# Autodesk Inventor assembly: Złożenie
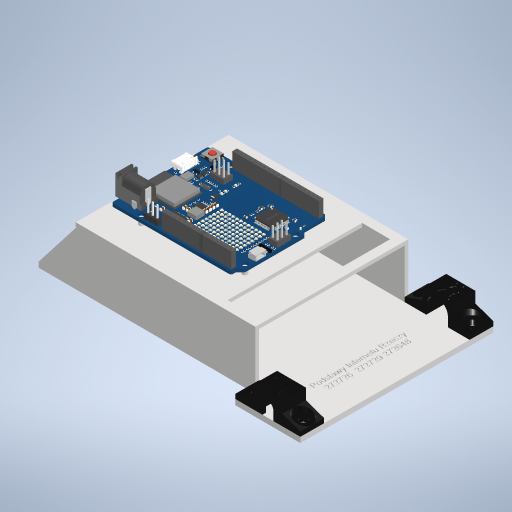
[picture p0: Inventor's stored thumbnail of the model, 512x512]
Saved by Autodesk Inventor 2024 (Build 280153020, 153B)
## iProperties
Created: 2025-01-23
Part Number: Złożenie
Document SubType Name: Assembly
Designer: jakub
Author: jakub
## Documents named in this file (4)
- C:\Users\jakub\OneDrive\Pulpit\Mikołaj wydruk\Złożenie.iam
- C:\Users\jakub\OneDrive\Pulpit\Mikołaj wydruk\Część1.ipt
- C:\Users\jakub\OneDrive\Pulpit\Mikołaj wydruk\N20.ipt
- C:\Users\jakub\OneDrive\Pulpit\Mikołaj wydruk\UNO R4 WiFi\UNO R4 WiFi.iam
## Components (4 placed, 3 different names)
1. Część1:1 — Zestawiające:1, Zestawiające:2, Zestawiające:6, Zestawiające:7, Zestawiające:8, Zestawiające:9, Zestawiające:10, Zestawiające:11, Zestawiające:12
2. N20:1 — Zestawiające:1, Zestawiające:8, Zestawiające:9
3. N20:2 — Zestawiające:2, Zestawiające:6, Zestawiające:7
4. UNO R4 WiFi:1 [sub-assembly] — Zestawiające:10, Zestawiające:11, Zestawiające:12
## Relationships (9: Mate 9)
- Zestawiające:1 [Mate]: Część1:1 ↔ N20:1
- Zestawiające:2 [Mate]: Część1:1 ↔ N20:2
- Zestawiające:6 [Mate]: Część1:1 ↔ N20:2
- Zestawiające:7 [Mate]: Część1:1 ↔ N20:2
- Zestawiające:8 [Mate]: Część1:1 ↔ N20:1
- Zestawiające:9 [Mate]: Część1:1 ↔ N20:1
- Zestawiające:10 [Mate]: Część1:1 ↔ UNO R4 WiFi:1
- Zestawiające:11 [Mate]: Część1:1 ↔ UNO R4 WiFi:1
- Zestawiające:12 [Mate]: Część1:1 ↔ UNO R4 WiFi:1
